# Autodesk Inventor assembly: Assembly1
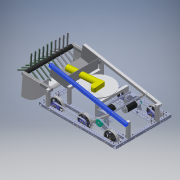
[picture p0: Inventor's stored thumbnail of the model, 180x180]
Saved by Autodesk Inventor 2016 (Build 200138000, 138)
## iProperties
Created: 2016-09-04
Part Number: Assembly1
Document SubType Name: Assembly
Designer: gus
Author: gus
## Documents named in this file (20)
- \\Mac\Home\Desktop\bunnybots 2016\1510_2898-16-Bunnybot-CAD\Design Ideas\prototype 002\Assembly1.iam
- \\Mac\Home\Desktop\bunnybots 2016\1510_2898-16-Bunnybot-CAD\Design Ideas\prototype 002\C-Base2LongTBMini6HiGripBelts.iam
- \\Mac\Home\Desktop\bunnybots 2016\1510_2898-16-Bunnybot-CAD\Design Ideas\prototype 002\Part88.ipt
- \\Mac\Home\Desktop\bunnybots 2016\1510_2898-16-Bunnybot-CAD\Design Ideas\prototype 002\Part89.ipt
- \\Mac\Home\Desktop\bunnybots 2016\1510_2898-16-Bunnybot-CAD\Design Ideas\prototype 002\Part88_MIR.ipt
- \\Mac\Home\Desktop\bunnybots 2016\1510_2898-16-Bunnybot-CAD\Design Ideas\prototype 002\Part89_MIR.ipt
- \\Mac\Home\Desktop\bunnybots 2016\1510_2898-16-Bunnybot-CAD\Design Ideas\prototype 002\Part93.ipt
- \\Mac\Home\Desktop\bunnybots 2016\1510_2898-16-Bunnybot-CAD\Design Ideas\prototype 002\Part95.ipt
- \\Mac\Home\Desktop\bunnybots 2016\1510_2898-16-Bunnybot-CAD\Design Ideas\prototype 002\Part1.ipt
- \\Mac\Home\Desktop\bunnybots 2016\1510_2898-16-Bunnybot-CAD\Design Ideas\prototype 002\Part2.ipt
- \\Mac\Home\Desktop\bunnybots 2016\1510_2898-16-Bunnybot-CAD\Design Ideas\prototype 002\Part1_MIR.ipt
- \\Mac\Home\Desktop\bunnybots 2016\1510_2898-16-Bunnybot-CAD\Design Ideas\prototype 002\Part2_MIR.ipt
- \\Mac\Home\Desktop\bunnybots 2016\1510_2898-16-Bunnybot-CAD\Design Ideas\prototype 002\Part4.ipt
- \\Mac\Home\Desktop\bunnybots 2016\1510_2898-16-Bunnybot-CAD\Design Ideas\prototype 002\Part100.ipt
- \\Mac\Home\Desktop\bunnybots 2016\1510_2898-16-Bunnybot-CAD\Design Ideas\prototype 002\part101.ipt
- \\Mac\Home\Desktop\bunnybots 2016\1510_2898-16-Bunnybot-CAD\Design Ideas\prototype 002\Part102.ipt
- \\Mac\Home\Desktop\bunnybots 2016\1510_2898-16-Bunnybot-CAD\Design Ideas\prototype 002\part104.ipt
- \\Mac\Home\Desktop\bunnybots 2016\1510_2898-16-Bunnybot-CAD\Design Ideas\prototype 002\Part88_MIR1.ipt
- \\Mac\Home\Desktop\bunnybots 2016\1510_2898-16-Bunnybot-CAD\Design Ideas\prototype 002\part104_MIR.ipt
- \\Mac\Home\Desktop\bunnybots 2016\1510_2898-16-Bunnybot-CAD\Design Ideas\prototype 002\Part5.ipt
## Components (50 placed, 19 different names)
1. C-Base2LongTBMini6HiGripBelts:1 [sub-assembly] — Flush:4, Mate:2, Mate:3, Flush:7, Flush:8, Mate:8, Tangent:2, Mate:13, Tangent:3, Mate:14, Mate:18, Mate:19, Mate:20, Flush:15, Mate:25, Flush:16, Flush:17, Mate:29, Flush:20
2. Part88:2 — Flush:4, Mate:2, Flush:5, Cylindrical:1, Mate:3, Flush:9, Flush:20
3. Part89:1 — Flush:5, Cylindrical:1, Cylindrical:10, Mate:16, Mate:17
4. Part88_MIR:1 — Mate:7, Cylindrical:2, Flush:8, Flush:9, Mate:8
5. Part89_MIR:1 — Mate:7, Cylindrical:2, Cylindrical:7, Mate:16, Mate:33, Flush:24, Flush:25
6. Part93:1 — Mate:10, Mate:11, Tangent:1, Cylindrical:12, Mate:27
7. Part1:1 — Cylindrical:4, Tangent:2, Mate:13
8. Part2:1 — Cylindrical:4, Cylindrical:7
9. Part1_MIR:1 — Cylindrical:8, Tangent:3, Mate:14
10. Part2_MIR:1 — Cylindrical:8, Cylindrical:10
11. Part4:1 — Mate:31, Mate:32, Flush:23
12. Part100:1 — Flush:12, Flush:13, Mate:18, Mate:20, Mate:21, Tangent:4
13. Part100:2 — Flush:12, Flush:13, Mate:17, Mate:19
14. part101:1 — Mate:21, Tangent:4, Mate:22, Mate:23, Mate:24
15. Part102:1 — Mate:23, Mate:24
16. Part88:3 — Flush:15, Mate:25, Flush:16, Cylindrical:11, Mate:26, Flush:18
17. part104:1 — Cylindrical:11, Mate:26, Cylindrical:12, Mate:27, Flush:19, Flush:22, Mate:31
18. Part88_MIR1:1 — Mate:28, Flush:17, Mate:29, Flush:18
19. part104_MIR:1 — Mate:28, Flush:19, Flush:22, Mate:32, Flush:23
20. Part5:1 — Mate:33, Flush:24, Flush:25
21. Part95:1 — Mate:10, Mate:11, Tangent:1
22. Part95:2
23. Part95:3
24. Part95:4
25. Part95:5
26. Part95:6
27. Part95:19
28. Part95:20
29. Part95:21
30. Part95:22
31. Part95:7
32. Part95:8
33. Part95:9
34. Part95:10
35. Part95:11
36. Part95:12
37. Part95:23
38. Part95:24
39. Part95:25
40. Part95:26
41. Part95:13
42. Part95:14
43. Part95:15
44. Part95:16
45. Part95:17
46. Part95:18
47. Part95:27
48. Part95:28
49. Part95:29
50. Part95:30
## Component patterns: (3 elements), (10 elements, first: Part95:1), Component Pattern 1:2 (10 elements), Component Pattern 1:3 (10 elements)
## Relationships (54: Mate 25, Flush 17, CylindricalJoint 8, Tangent 4)
- Flush:4: C-Base2LongTBMini6HiGripBelts:1 ↔ Part88:2
- Mate:2: C-Base2LongTBMini6HiGripBelts:1 ↔ Part88:2
- Flush:5: Part88:2 ↔ Part89:1
- Cylindrical:1: Part88:2 ↔ Part89:1
- Mate:3: C-Base2LongTBMini6HiGripBelts:1 ↔ Part88:2
- Flush:7 (-292.1 mm): C-Base2LongTBMini6HiGripBelts:1
- Mate:7: Part88_MIR:1 ↔ Part89_MIR:1
- Cylindrical:2: Part88_MIR:1 ↔ Part89_MIR:1
- Flush:8: C-Base2LongTBMini6HiGripBelts:1 ↔ Part88_MIR:1
- Flush:9: Part88:2 ↔ Part88_MIR:1
- Mate:8: C-Base2LongTBMini6HiGripBelts:1 ↔ Part88_MIR:1
- Mate:10: Part93:1 ↔ Part95:1
- Mate:11: Part93:1 ↔ Part95:1
- Tangent:1 (50.8 mm): Part93:1 ↔ Part95:1
- Cylindrical:4: Part1:1 ↔ Part2:1
- Tangent:2: C-Base2LongTBMini6HiGripBelts:1 ↔ Part1:1
- Cylindrical:7: Part89_MIR:1 ↔ Part2:1
- Cylindrical:8: Part1_MIR:1 ↔ Part2_MIR:1
- Cylindrical:10: Part89:1 ↔ Part2_MIR:1
- Mate:13: C-Base2LongTBMini6HiGripBelts:1 ↔ Part1:1
- Tangent:3: C-Base2LongTBMini6HiGripBelts:1 ↔ Part1_MIR:1
- Mate:14: C-Base2LongTBMini6HiGripBelts:1 ↔ Part1_MIR:1
- Mate:16: Part89:1 ↔ Part89_MIR:1
- Flush:12: Part100:1 ↔ Part100:2
- Flush:13: Part100:1 ↔ Part100:2
- Mate:17: Part89:1 ↔ Part100:2
- Mate:18: C-Base2LongTBMini6HiGripBelts:1 ↔ Part100:1
- Mate:19: C-Base2LongTBMini6HiGripBelts:1 ↔ Part100:2
- Mate:20: C-Base2LongTBMini6HiGripBelts:1 ↔ Part100:1
- Mate:21: Part100:1 ↔ part101:1
- Tangent:4: Part100:1 ↔ part101:1
- Mate:22: part101:1
- Mate:23: part101:1 ↔ Part102:1
- Mate:24: part101:1 ↔ Part102:1
- Flush:15: C-Base2LongTBMini6HiGripBelts:1 ↔ Part88:3
- Mate:25: C-Base2LongTBMini6HiGripBelts:1 ↔ Part88:3
- Flush:16 (76.2 mm): C-Base2LongTBMini6HiGripBelts:1 ↔ Part88:3
- Cylindrical:11: Part88:3 ↔ part104:1
- Mate:26: Part88:3 ↔ part104:1
- Cylindrical:12: Part93:1 ↔ part104:1
- Mate:27: Part93:1 ↔ part104:1
- Mate:28: Part88_MIR1:1 ↔ part104_MIR:1
- Flush:17: C-Base2LongTBMini6HiGripBelts:1 ↔ Part88_MIR1:1
- Mate:29: C-Base2LongTBMini6HiGripBelts:1 ↔ Part88_MIR1:1
- Flush:18: Part88:3 ↔ Part88_MIR1:1
- Flush:19: part104:1 ↔ part104_MIR:1
- Flush:20: C-Base2LongTBMini6HiGripBelts:1 ↔ Part88:2
- Flush:22: part104:1 ↔ part104_MIR:1
- Mate:31: Part4:1 ↔ part104:1
- Mate:32: Part4:1 ↔ part104_MIR:1
- Flush:23: Part4:1 ↔ part104_MIR:1
- Mate:33: Part89_MIR:1 ↔ Part5:1
- Flush:24: Part89_MIR:1 ↔ Part5:1
- Flush:25: Part89_MIR:1 ↔ Part5:1
